# Autodesk Inventor assembly: 部件1
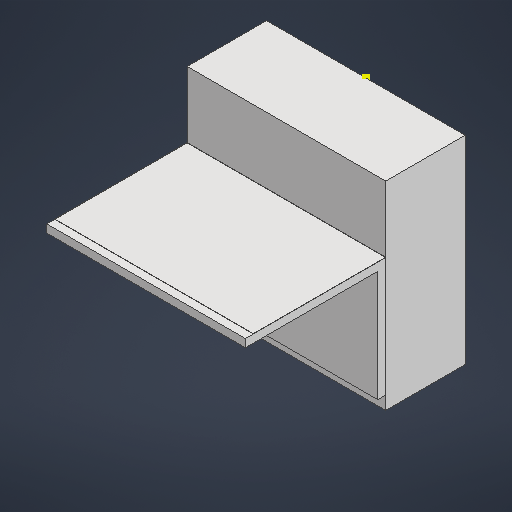
[picture p0: Inventor's stored thumbnail of the model, 512x512]
Saved by Autodesk Inventor 2025 (Build 290162000, 162)
## iProperties
Created: 2025-11-30
Part Number: 部件1
Document SubType Name: Assembly
Designer: XH
Author: XH
## Documents named in this file (3)
- D:\盲文打印机\部件1.iam
- D:\盲文打印机\便签.ipt
- D:\盲文打印机\主体.ipt
## Components (2 placed, 2 different names)
1. 便签:1 — 配合:1, 表面齐平:1, 配合:2
2. 主体:1 — 配合:1, 表面齐平:1, 配合:2
## Relationships (3: Mate 2, Flush 1)
- 配合:1 [Mate]: 便签:1 ↔ 主体:1
- 表面齐平:1 [Flush]: 便签:1 ↔ 主体:1
- 配合:2 [Mate]: 便签:1 ↔ 主体:1
